# Autodesk Inventor assembly: Baugruppe Fliegenfalle
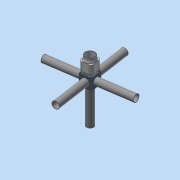
[picture p0: Inventor's stored thumbnail of the model, 180x180]
Saved by Autodesk Inventor 2019 (Build 230136000, 136)
## iProperties
Created: 2019-03-27
Part Number: Baugruppe Fliegenfalle
Material: Generisch
Document SubType Name: Assembly
Designer: Martin
Author: Martin
## Documents named in this file (5)
- C:\Feinmechanik ab 2015\Renz\Fliegenfalle\Baugruppe Fliegenfalle.iam
- C:\Feinmechanik ab 2015\Renz\Fliegenfalle\Block.ipt
- C:\Feinmechanik ab 2015\Renz\Fliegenfalle\Rohr.ipt
- C:\Feinmechanik ab 2015\Renz\Fliegenfalle\Baugruppe Schraube.iam
- C:\Feinmechanik ab 2015\Renz\Fliegenfalle\Lüfter.ipt
## Components (11 placed, 4 different names)
1. Block:1 — Starr:1, Drehbar:1, Starr:2, Starr:3, Passend:1, Drehbar:2, Drehbar:3, Drehbar:4, Passend:2, Passend:3, Passend:4, Passend:5, Winkel:1
2. Rohr:1 — Drehbar:1
3. Rohr:2 — Starr:3
4. Rohr:3 — Starr:2
5. Rohr:4 — Starr:1
6. Baugruppe Schraube:1 [sub-assembly] — Drehbar:2
7. Baugruppe Schraube:2 [sub-assembly] — Drehbar:3
8. Baugruppe Schraube:3 [sub-assembly] — Drehbar:4
9. Baugruppe Schraube:4 [sub-assembly] — Passend:1
10. Rohr:5 — Passend:2, Passend:3
11. Lüfter:1 — Passend:4, Passend:5, Winkel:1
## Relationships (13: Mate 5, RevoluteJoint 4, WeldJoint 3, Angle 1)
- Starr:1 [WeldJoint]: Block:1 ↔ Rohr:4
- Drehbar:1 [RevoluteJoint]: Block:1 ↔ Rohr:1
- Starr:2 [WeldJoint]: Block:1 ↔ Rohr:3
- Starr:3 [WeldJoint]: Block:1 ↔ Rohr:2
- Passend:1 [Mate]: Block:1 ↔ Baugruppe Schraube:4
- Drehbar:2 [RevoluteJoint]: Block:1 ↔ Baugruppe Schraube:1
- Drehbar:3 [RevoluteJoint]: Block:1 ↔ Baugruppe Schraube:2
- Drehbar:4 [RevoluteJoint]: Block:1 ↔ Baugruppe Schraube:3
- Passend:2 [Mate]: Block:1 ↔ Rohr:5
- Passend:3 [Mate]: Block:1 ↔ Rohr:5
- Passend:4 [Mate]: Block:1 ↔ Lüfter:1
- Passend:5 [Mate]: Block:1 ↔ Lüfter:1
- Winkel:1 [Angle] (0 deg): Block:1 ↔ Lüfter:1
